# Autodesk Inventor assembly: ASM_Micron_ASAP_Indep60
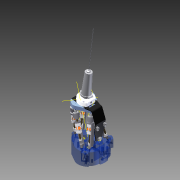
[picture p0: Inventor's stored thumbnail of the model, 180x180]
Saved by Autodesk Inventor 2011 SP2 (Build 150309200, 309)
## iProperties
Created: 2011-08-12
Part Number: ASM_Micron_ASAP_Indep60
Document SubType Name: Assembly
Designer: sungwook
Author: sungwook
## Documents named in this file (10)
- C:\Users\sungwook\Documents\Inventor\Micron20_Base_Tube_Adjst\Assembly\Motion_Merge\ASM_Micron_ASAP_Indep60.iam
- C:\Users\sungwook\Documents\Inventor\Micron20_Base_Tube_Adjst\Parts\Main\Platform_Base_20mm_Rev2.ipt
- C:\Users\sungwook\Documents\Inventor\Micron20_Base_Tube_Adjst\Parts\Main\Platform_Top_14mm_Rev.ipt
- C:\Users\sungwook\Documents\Inventor\Micron20_Base_Tube_Adjst\Parts\Tool\ASM_Tool_Tip_Rev.iam
- C:\Users\sungwook\Documents\Inventor\Micron20_Base_Tube_Adjst\Assembly\ASM_Motor_Unit_Part1_Rev.iam
- C:\Users\sungwook\Documents\Inventor\Micron20_Base_Tube_Adjst\Assembly\ASM_Motor_Unit_Part2_Rev.iam
- C:\Users\sungwook\Documents\Inventor\Micron20_Base_Tube_Adjst\Parts\ASAP\Platform_ASAP.iam
- C:\Users\sungwook\Documents\Inventor\Micron20_Base_Tube_Adjst\Parts\Main\Spring.ipt
- C:\Users\sungwook\Documents\Inventor\Micron20_Base_Tube_Adjst\Parts\Main\Eye_Pin_26Ga.ipt
- C:\Users\sungwook\Documents\Inventor\Micron20_Base_Tube_Adjst\Param_dMotor.xlsx
## Components (25 placed, 8 different names)
1. Platform_Base_20mm_Rev2:1 — Angle_Top_Bottom, Mate_Top_Bottom, Top_Bottom_Default, Mate:46, Mate:47, Mate:48, Mate:49, Mate:50, Mate:51, Mate:81, Mate:82
2. Platform_Top_14mm_Rev:1 — Angle_Top_Bottom, Mate_Top_Bottom, Mate:20, Mate:21, Mate:22, Top_Bottom_Default, Mate:58, Mate:59, Mate:60, Mate:61, Mate:62, Mate:63, Mate:72, Mate:73, Mate:74, Mate:76, Flush:1, Angle:8, Mate:94, Flush:2, Mate:95, Flush:3
3. ASM_Tool_Tip_Rev:1 [sub-assembly] — Mate:20, Mate:21, Mate:22, Mate:73, Mate:70
4. ASM_Motor_Unit_Part1_Rev:1 [sub-assembly] — Mate:46, Mate:52, Angle:5, Mate:64
5. ASM_Motor_Unit_Part2_Rev:1 [sub-assembly] — Mate:52, Mate:58, Mate:64
6. ASM_Motor_Unit_Part1_Rev:2 [sub-assembly] — Mate:47, Mate:53, Angle:6, Mate:65
7. ASM_Motor_Unit_Part2_Rev:2 [sub-assembly] — Mate:53, Mate:59, Mate:65
8. ASM_Motor_Unit_Part1_Rev:3 [sub-assembly] — Mate:48, Mate:54, Angle:6, Mate:66
9. ASM_Motor_Unit_Part2_Rev:3 [sub-assembly] — Mate:54, Mate:60, Mate:66
10. ASM_Motor_Unit_Part1_Rev:4 [sub-assembly] — Mate:49, Mate:55, Angle:7, Mate:67
11. ASM_Motor_Unit_Part2_Rev:4 [sub-assembly] — Mate:55, Mate:61, Mate:67
12. ASM_Motor_Unit_Part1_Rev:5 [sub-assembly] — Mate:50, Mate:56, Angle:7, Mate:68
13. ASM_Motor_Unit_Part2_Rev:5 [sub-assembly] — Mate:56, Mate:62, Mate:68
14. ASM_Motor_Unit_Part1_Rev:6 [sub-assembly] — Mate:51, Mate:57, Angle:5, Mate:69
15. ASM_Motor_Unit_Part2_Rev:6 [sub-assembly] — Mate:57, Mate:63, Mate:69
16. Platform_ASAP:1 [sub-assembly] — Mate:70, Mate:72, Mate:74
17. Spring:1 — Mate:77, Mate:88, Mate:89
18. Spring:2 — Mate:90, Mate:92
19. Spring:3 — Mate:91, Mate:93
20. Eye_Pin_26Ga:4 — Mate:83, Mate:92, Mate:95, Flush:3
21. Eye_Pin_26Ga:5 — Mate:85, Mate:93, Mate:94, Flush:2
22. Eye_Pin_26Ga:1 — Mate:76, Flush:1, Angle:8, Mate:77
23. Eye_Pin_26Ga:6 — Mate:81, Mate:82, Mate:87
24. Eye_Pin_26Ga:7 — Mate:84
25. Eye_Pin_26Ga:8 — Mate:86
## Component patterns: (3 elements, first: Eye_Pin_26Ga:1), (3 elements, first: Eye_Pin_26Ga:6)
## Relationships (58: Mate 50, Angle 5, Flush 3)
- Angle_Top_Bottom (0 deg): Platform_Base_20mm_Rev2:1 ↔ Platform_Top_14mm_Rev:1
- Mate_Top_Bottom (30 mm): Platform_Base_20mm_Rev2:1 ↔ Platform_Top_14mm_Rev:1
- Mate:20: Platform_Top_14mm_Rev:1 ↔ ASM_Tool_Tip_Rev:1
- Mate:21: Platform_Top_14mm_Rev:1 ↔ ASM_Tool_Tip_Rev:1
- Mate:22: Platform_Top_14mm_Rev:1 ↔ ASM_Tool_Tip_Rev:1
- Top_Bottom_Default [Mate] (26.2836 mm): Platform_Base_20mm_Rev2:1 ↔ Platform_Top_14mm_Rev:1
- Mate:46: Platform_Base_20mm_Rev2:1 ↔ ASM_Motor_Unit_Part1_Rev:1
- Mate:47: Platform_Base_20mm_Rev2:1 ↔ ASM_Motor_Unit_Part1_Rev:2
- Mate:48: Platform_Base_20mm_Rev2:1 ↔ ASM_Motor_Unit_Part1_Rev:3
- Mate:49: Platform_Base_20mm_Rev2:1 ↔ ASM_Motor_Unit_Part1_Rev:4
- Mate:50: Platform_Base_20mm_Rev2:1 ↔ ASM_Motor_Unit_Part1_Rev:5
- Mate:51: Platform_Base_20mm_Rev2:1 ↔ ASM_Motor_Unit_Part1_Rev:6
- Mate:52: ASM_Motor_Unit_Part1_Rev:1 ↔ ASM_Motor_Unit_Part2_Rev:1
- Mate:53: ASM_Motor_Unit_Part1_Rev:2 ↔ ASM_Motor_Unit_Part2_Rev:2
- Mate:54: ASM_Motor_Unit_Part1_Rev:3 ↔ ASM_Motor_Unit_Part2_Rev:3
- Mate:55: ASM_Motor_Unit_Part1_Rev:4 ↔ ASM_Motor_Unit_Part2_Rev:4
- Mate:56: ASM_Motor_Unit_Part1_Rev:5 ↔ ASM_Motor_Unit_Part2_Rev:5
- Mate:57: ASM_Motor_Unit_Part1_Rev:6 ↔ ASM_Motor_Unit_Part2_Rev:6
- Mate:58: Platform_Top_14mm_Rev:1 ↔ ASM_Motor_Unit_Part2_Rev:1
- Mate:59: Platform_Top_14mm_Rev:1 ↔ ASM_Motor_Unit_Part2_Rev:2
- Mate:60: Platform_Top_14mm_Rev:1 ↔ ASM_Motor_Unit_Part2_Rev:3
- Mate:61: Platform_Top_14mm_Rev:1 ↔ ASM_Motor_Unit_Part2_Rev:4
- Mate:62: Platform_Top_14mm_Rev:1 ↔ ASM_Motor_Unit_Part2_Rev:5
- Mate:63: Platform_Top_14mm_Rev:1 ↔ ASM_Motor_Unit_Part2_Rev:6
- Angle:5 (180 deg): ASM_Motor_Unit_Part1_Rev:1 ↔ ASM_Motor_Unit_Part1_Rev:6
- Angle:6 (180 deg): ASM_Motor_Unit_Part1_Rev:2 ↔ ASM_Motor_Unit_Part1_Rev:3
- Angle:7 (180 deg): ASM_Motor_Unit_Part1_Rev:4 ↔ ASM_Motor_Unit_Part1_Rev:5
- Mate:64 (0.344 mm): ASM_Motor_Unit_Part1_Rev:1 ↔ ASM_Motor_Unit_Part2_Rev:1
- Mate:65 (1.989 mm): ASM_Motor_Unit_Part1_Rev:2 ↔ ASM_Motor_Unit_Part2_Rev:2
- Mate:66 (0.848 mm): ASM_Motor_Unit_Part1_Rev:3 ↔ ASM_Motor_Unit_Part2_Rev:3
- Mate:67 (0.848 mm): ASM_Motor_Unit_Part1_Rev:4 ↔ ASM_Motor_Unit_Part2_Rev:4
- Mate:68 (1.989 mm): ASM_Motor_Unit_Part1_Rev:5 ↔ ASM_Motor_Unit_Part2_Rev:5
- Mate:69 (0.344 mm): ASM_Motor_Unit_Part1_Rev:6 ↔ ASM_Motor_Unit_Part2_Rev:6
- Mate:70: ASM_Tool_Tip_Rev:1 ↔ Platform_ASAP:1
- Mate:72: Platform_Top_14mm_Rev:1 ↔ Platform_ASAP:1
- Mate:73: Platform_Top_14mm_Rev:1 ↔ ASM_Tool_Tip_Rev:1
- Mate:74: Platform_Top_14mm_Rev:1 ↔ Platform_ASAP:1
- Mate:76: Platform_Top_14mm_Rev:1 ↔ Eye_Pin_26Ga:1
- Flush:1: Platform_Top_14mm_Rev:1 ↔ Eye_Pin_26Ga:1
- Angle:8 (0 deg): Platform_Top_14mm_Rev:1 ↔ Eye_Pin_26Ga:1
- Mate:77: Spring:1 ↔ Eye_Pin_26Ga:1
- Mate:81: Platform_Base_20mm_Rev2:1 ↔ Eye_Pin_26Ga:6
- Mate:82: Platform_Base_20mm_Rev2:1 ↔ Eye_Pin_26Ga:6
- Mate:83: Eye_Pin_26Ga:4
- Mate:84: Eye_Pin_26Ga:7
- Mate:85: Eye_Pin_26Ga:5
- Mate:86: Eye_Pin_26Ga:8
- Mate:87: Eye_Pin_26Ga:6
- Mate:88: Spring:1
- Mate:89: Spring:1
- Mate:90: Spring:2
- Mate:91: Spring:3
- Mate:92: Spring:2 ↔ Eye_Pin_26Ga:4
- Mate:93: Spring:3 ↔ Eye_Pin_26Ga:5
- Mate:94: Platform_Top_14mm_Rev:1 ↔ Eye_Pin_26Ga:5
- Flush:2: Platform_Top_14mm_Rev:1 ↔ Eye_Pin_26Ga:5
- Mate:95: Platform_Top_14mm_Rev:1 ↔ Eye_Pin_26Ga:4
- Flush:3: Platform_Top_14mm_Rev:1 ↔ Eye_Pin_26Ga:4
## Named parameters: dMotor1 = 0.344 mm, dMotor2 = 1.989 mm, dMotor3 = 0.848 mm, dMotor4 = 0.848 mm, dMotor5 = 1.989 mm, dMotor6 = 0.344 mm
